# Autodesk Inventor assembly: Case_Assembly
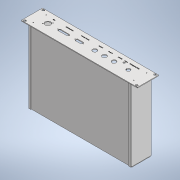
[picture p0: Inventor's stored thumbnail of the model, 180x180]
Saved by Autodesk Inventor 2022.2 (Build 262287010, 287A)
## iProperties
Created: 2024-11-06
Part Number: Case_Assembly
Document SubType Name: Assembly
Designer: ppovolni
Author: ppovolni
## Documents named in this file (5)
- M:\3_Projekte\3_LowFieldScanner\4_Messrobotik und Sensorik\Bumblebee_OpenSource\Hardware\Case\Case_Assembly.iam
- M:\3_Projekte\3_LowFieldScanner\4_Messrobotik und Sensorik\Bumblebee_OpenSource\Hardware\Case\Case_Front.ipt
- M:\3_Projekte\3_LowFieldScanner\4_Messrobotik und Sensorik\Bumblebee_OpenSource\Hardware\Case\Case_Side.ipt
- M:\3_Projekte\3_LowFieldScanner\4_Messrobotik und Sensorik\Bumblebee_OpenSource\Hardware\Case\Case_Back.ipt
- M:\3_Projekte\3_LowFieldScanner\4_Messrobotik und Sensorik\Bumblebee_OpenSource\Hardware\Case\Case_Top.ipt
## Components (5 placed, 4 different names)
1. Case_Front:1 — Passend:1, Passend:2, Winkel:1, Passend:3, Passend:4, Winkel:2, Fluchtend:3, Fluchtend:4
2. Case_Side:1 — Passend:1, Passend:2, Winkel:1, Fluchtend:1
3. Case_Side:2 — Passend:3, Passend:4, Winkel:2, Fluchtend:2
4. Case_Back:1 — Fluchtend:1, Fluchtend:2
5. Case_Top:1 — Fluchtend:3, Fluchtend:4
## Relationships (10: Mate 4, Flush 4, Angle 2)
- Passend:1 [Mate]: Case_Front:1 ↔ Case_Side:1
- Passend:2 [Mate]: Case_Front:1 ↔ Case_Side:1
- Winkel:1 [Angle] (0 deg): Case_Front:1 ↔ Case_Side:1
- Passend:3 [Mate]: Case_Front:1 ↔ Case_Side:2
- Passend:4 [Mate]: Case_Front:1 ↔ Case_Side:2
- Winkel:2 [Angle] (0 deg): Case_Front:1 ↔ Case_Side:2
- Fluchtend:1 [Flush]: Case_Side:1 ↔ Case_Back:1
- Fluchtend:2 [Flush]: Case_Side:2 ↔ Case_Back:1
- Fluchtend:3 [Flush]: Case_Front:1 ↔ Case_Top:1
- Fluchtend:4 [Flush]: Case_Front:1 ↔ Case_Top:1
